# Autodesk Inventor assembly: platform_0606_fig2_ratio10
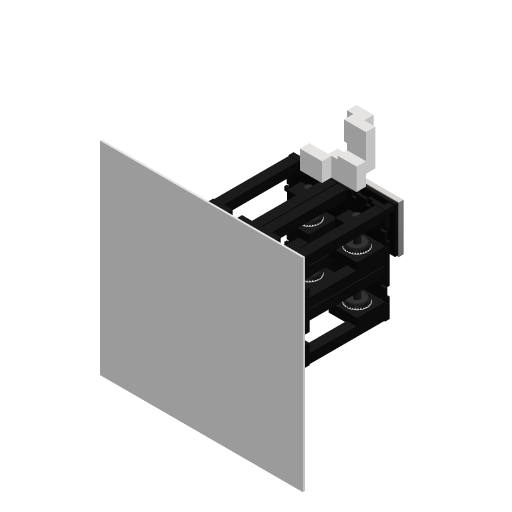
[picture p0: Inventor's stored thumbnail of the model, 512x512]
Saved by Autodesk Inventor 2024 (Build 280153000, 153)
## iProperties
Created: 2024-06-06
Part Number: platform_0606_fig2_ratio10
Document SubType Name: Assembly
Designer: admin
Author: admin
## Documents named in this file (8)
- C:\Users\admin\OneDrive\文件\碩士研究\prototype\plane_unit_0606\platform_0606_fig2_ladder.iam
- C:\Users\admin\OneDrive\文件\碩士研究\prototype\plane_unit_0606\one_way_bearing.ipt
- C:\Users\admin\OneDrive\文件\碩士研究\prototype\plane_unit_0606\printer_base_plane.ipt
- C:\Users\admin\OneDrive\文件\碩士研究\prototype\plane_unit_0606\rod_1221.ipt
- C:\Users\admin\OneDrive\文件\碩士研究\prototype\plane_unit_0606\iron_plate.ipt
- C:\Users\admin\OneDrive\文件\碩士研究\prototype\plane_unit_0606\plane_unit_1121.ipt
- C:\Users\admin\OneDrive\文件\碩士研究\prototype\plane_unit_0606\gear_pin_1222_.ipt
- C:\Users\admin\OneDrive\文件\碩士研究\prototype\plane_unit_0606\Template_ladder_2.ipt
## Components (16 placed, 7 different names)
1. printer_base_plane:1 — 貼合:1, 齊平:1, 齊平:2, 齊平:4
2. rod_1221:1 — 貼合:7, 貼合:8, 貼合:9, 貼合:10, 貼合:11
3. iron_plate:1 — 貼合:9, 貼合:10, 貼合:11, 齊平:4
4. Template_ladder_2:1
5. one_way_bearing:1 — 貼合:2, 齊平:3, 貼合:3, 貼合:4
6. plane_unit_1121:1 — 貼合:1, 齊平:1, 齊平:2, 貼合:2, 齊平:3, 貼合:7, 貼合:8
7. gear_pin_1222_:1 — 貼合:3, 貼合:4
8. one_way_bearing:2
9. plane_unit_1121:2
10. gear_pin_1222_:2
11. one_way_bearing:3
12. plane_unit_1121:3
13. gear_pin_1222_:3
14. one_way_bearing:4
15. plane_unit_1121:4
16. gear_pin_1222_:4
## Component patterns: (4 elements, first: one_way_bearing:1 + plane_unit_1121:1 + gear_pin_1222_:1)
## Relationships (13: Mate 9, Flush 4)
- 貼合:1 [Mate]: printer_base_plane:1 ↔ plane_unit_1121:1
- 齊平:1 [Flush] (5 mm): printer_base_plane:1 ↔ plane_unit_1121:1
- 齊平:2 [Flush] (5 mm): printer_base_plane:1 ↔ plane_unit_1121:1
- 貼合:2 [Mate]: one_way_bearing:1 ↔ plane_unit_1121:1
- 齊平:3 [Flush]: one_way_bearing:1 ↔ plane_unit_1121:1
- 貼合:3 [Mate]: one_way_bearing:1 ↔ gear_pin_1222_:1
- 貼合:4 [Mate]: one_way_bearing:1 ↔ gear_pin_1222_:1
- 貼合:7 [Mate] (0.2 mm): rod_1221:1 ↔ plane_unit_1121:1
- 貼合:8 [Mate] (0.2 mm): rod_1221:1 ↔ plane_unit_1121:1
- 貼合:9 [Mate]: rod_1221:1 ↔ iron_plate:1
- 貼合:10 [Mate]: rod_1221:1 ↔ iron_plate:1
- 貼合:11 [Mate]: rod_1221:1 ↔ iron_plate:1
- 齊平:4 [Flush] (-110 mm): printer_base_plane:1 ↔ iron_plate:1
